# Autodesk Inventor assembly: X_CarriageR_V2_0
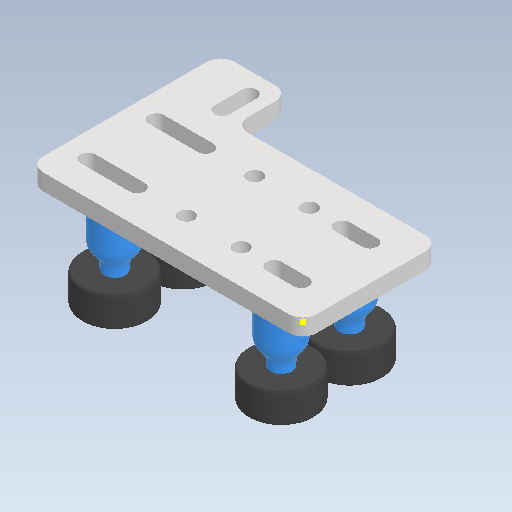
[picture p0: Inventor's stored thumbnail of the model, 512x512]
Saved by Autodesk Inventor 2021 (Build 250183000, 183)
## iProperties
Created: 2021-06-13
Part Number: X_CarriageR_V2_0
Document SubType Name: Assembly
Designer: Jorian Brusind
Author: Jorian Brusind
## Documents named in this file (6)
- C:\Users\Jorian Bruslind\Documents\GitHub\PersonalProjects\HyperRail\Inventor Files\X_CarriageR_V2_0.iam
- C:\Users\Jorian Bruslind\Documents\GitHub\PersonalProjects\HyperRail\Inventor Files\X_Carriage_Plate.ipt
- C:\Users\Jorian Bruslind\Documents\GitHub\PersonalProjects\HyperRail\Inventor Files\11mm_BearingWheel.ipt
- C:\Users\Jorian Bruslind\Documents\GitHub\PersonalProjects\HyperRail\Inventor Files\4mm_Roller_Spacer_simple.ipt
- C:\Users\Jorian Bruslind\Documents\GitHub\PersonalProjects\HyperRail\Inventor Files\Rollder_Spacer_Single.ipt
- C:\Users\Jorian Bruslind\Documents\GitHub\PersonalProjects\HyperRail\Inventor Files\10mm_Idle_Pulley.ipt
## Components (9 placed, 5 different names)
1. X_Carriage_Plate:1 — Mate:13, Mate:35, Mate:41, Mate:57, Mate:60, Angle:1, Angle:2, Mate:63
2. 11mm_BearingWheel:1 — Flush:2, Mate:62
3. 11mm_BearingWheel:4 — Flush:2, Mate:58, Mate:61
4. 4mm_Roller_Spacer_simple:1 — Mate:13, Mate:60, Angle:1, Mate:64, Mate:65, Mate:66
5. Rollder_Spacer_Single:1 — Mate:35, Mate:40, Mate:41, Mate:42
6. 10mm_Idle_Pulley:1 — Mate:40, Mate:42
7. 4mm_Roller_Spacer_simple:2 — Mate:57, Mate:58, Mate:61, Mate:62, Angle:2, Mate:63
8. 11mm_BearingWheel:5 — Mate:64, Flush:3
9. 11mm_BearingWheel:6 — Mate:65, Flush:3, Mate:66
## Relationships (18: Mate 14, Flush 2, Angle 2)
- Flush:2: 11mm_BearingWheel:1 ↔ 11mm_BearingWheel:4
- Mate:13: X_Carriage_Plate:1 ↔ 4mm_Roller_Spacer_simple:1
- Mate:35: X_Carriage_Plate:1 ↔ Rollder_Spacer_Single:1
- Mate:40: Rollder_Spacer_Single:1 ↔ 10mm_Idle_Pulley:1
- Mate:41: X_Carriage_Plate:1 ↔ Rollder_Spacer_Single:1
- Mate:42: Rollder_Spacer_Single:1 ↔ 10mm_Idle_Pulley:1
- Mate:57: X_Carriage_Plate:1 ↔ 4mm_Roller_Spacer_simple:2
- Mate:58: 11mm_BearingWheel:4 ↔ 4mm_Roller_Spacer_simple:2
- Mate:60 (-12.5 mm): X_Carriage_Plate:1 ↔ 4mm_Roller_Spacer_simple:1
- Angle:1 (0 deg): X_Carriage_Plate:1 ↔ 4mm_Roller_Spacer_simple:1
- Mate:61: 11mm_BearingWheel:4 ↔ 4mm_Roller_Spacer_simple:2
- Mate:62: 11mm_BearingWheel:1 ↔ 4mm_Roller_Spacer_simple:2
- Angle:2 (0 deg): X_Carriage_Plate:1 ↔ 4mm_Roller_Spacer_simple:2
- Mate:63 (-12.5 mm): X_Carriage_Plate:1 ↔ 4mm_Roller_Spacer_simple:2
- Mate:64: 4mm_Roller_Spacer_simple:1 ↔ 11mm_BearingWheel:5
- Mate:65: 4mm_Roller_Spacer_simple:1 ↔ 11mm_BearingWheel:6
- Flush:3: 11mm_BearingWheel:5 ↔ 11mm_BearingWheel:6
- Mate:66: 4mm_Roller_Spacer_simple:1 ↔ 11mm_BearingWheel:6
